# Autodesk Inventor assembly: Cover with Module
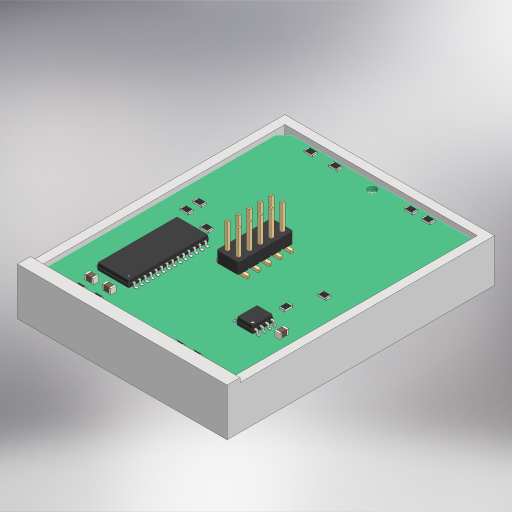
[picture p0: Inventor's stored thumbnail of the model, 512x512]
Saved by Autodesk Inventor 2024 (Build 280153000, 153)
## iProperties
Created: 2023-10-04
Part Number: Cover with Module
Document SubType Name: Assembly
Designer: cfang
Author: cfang
## Documents named in this file (3)
- C:\Users\cfang\Desktop\nebraska-silicon-lab\Hardware\ETL\modules\tamale v1.5 Thermal Mockup\Cover with Module.iam
- C:\Users\cfang\Desktop\nebraska-silicon-lab\Hardware\ETL\modules\tamale v1.5 Thermal Mockup\etl_module_pcb_thermal_mockup_v3\etl_module_pcb_thermal_mockup_v3.ipt
- C:\Users\cfang\Desktop\nebraska-silicon-lab\Hardware\ETL\modules\tamale v1.5 Thermal Mockup\Module Cover.ipt
## Components (2 placed, 2 different names)
1. etl_module_pcb_thermal_mockup_v3:1 — Mate:1, Mate:2
2. Module Cover:1 — Mate:1, Mate:2
## Relationships (2: Mate 2)
- Mate:1: etl_module_pcb_thermal_mockup_v3:1 ↔ Module Cover:1
- Mate:2: etl_module_pcb_thermal_mockup_v3:1 ↔ Module Cover:1
